# Autodesk Inventor assembly: Receiver Pins
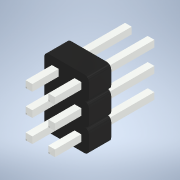
[picture p0: Inventor's stored thumbnail of the model, 180x180]
Saved by Autodesk Inventor 2020.1 (Build 241239000, 239)
## iProperties
Created: 2019-07-29
Part Number: Receiver Pins
Document SubType Name: Assembly
Designer: Petar
Author: Petar
## Documents named in this file (2)
- D:\OMG\E-Board\CAD\Inventor\Electrical Components\Receiver Pins.iam
- D:\OMG\E-Board\CAD\Inventor\Electrical Components\Arduino Nano\2pin_header__02.ipt
## Components (3 placed, 1 different names)
1. 2pin_header__02:1 — Rigid:1, Rigid:2
2. 2pin_header__02:2 — Rigid:2
3. 2pin_header__02:3 — Rigid:1
## Relationships (2: WeldJoint 2)
- Rigid:1 [WeldJoint]: 2pin_header__02:1 ↔ 2pin_header__02:3
- Rigid:2 [WeldJoint]: 2pin_header__02:1 ↔ 2pin_header__02:2
